# Autodesk Inventor assembly: hologram display version 2 assembly.ipt
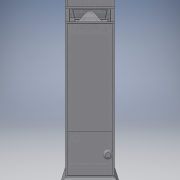
[picture p0: Inventor's stored thumbnail of the model, 180x180]
Saved by Autodesk Inventor 2016 (Build 200138000, 138)
## iProperties
Created: 2017-10-23
Part Number: hologram display version 2 assembly.ipt
Document SubType Name: Assembly
Designer: student
Author: student
## Documents named in this file (13)
- C:\Users\student\Documents\Aaron's Folder\hologram display version 2 assembly.ipt.iam
- C:\Users\student\Documents\Aaron's Folder\base (for assembly).ipt
- C:\Users\student\Documents\Aaron's Folder\support platforms (for assembly).ipt
- C:\Users\student\Documents\Aaron's Folder\side boards (for assembly).ipt
- C:\Users\student\Documents\Aaron's Folder\back board (for assembly).ipt
- C:\Users\student\Documents\Aaron's Folder\front board (for assembly).ipt
- C:\Users\student\Documents\Aaron's Folder\front door (for assembly).ipt
- C:\Users\student\Documents\Aaron's Folder\monitor supports (for assembly).ipt
- C:\Users\student\Documents\Aaron's Folder\monitor frame part1 (for assembly).ipt
- C:\Users\student\Documents\Aaron's Folder\monitor frame part2 (for assembly).ipt
- C:\Users\student\Documents\Aaron's Folder\hologram pyramid (for assembly).ipt
- C:\Users\student\Documents\Aaron's Folder\monitor (for assembly).ipt
- C:\Users\student\Documents\Aaron's Folder\hollow monitor support (for assembly).ipt
## Components (17 placed, 12 different names)
1. base (for assembly):1 — Rigid:1
2. support platforms (for assembly):1 — Rigid:1, Rigid:19, Rigid:29
3. side boards (for assembly):1 — Rigid:18, Rigid:29, Rigid:30
4. side boards (for assembly):2 — Rigid:18
5. support platforms (for assembly):2 — Rigid:19, Rigid:20, Rigid:21, Rigid:22, Rigid:24, Rigid:31
6. back board (for assembly):1 — Rigid:15, Rigid:16, Rigid:30
7. front board (for assembly):1 — Rigid:16
8. front door (for assembly):1 — Rigid:15
9. monitor supports (for assembly):2 — Rigid:21
10. monitor supports (for assembly):3 — Rigid:20, Rigid:25
11. monitor supports (for assembly):4 — Rigid:22
12. hologram pyramid (for assembly):1 — Rigid:24
13. monitor frame part1 (for assembly):1 — Rigid:25, Rigid:27, Rigid:32
14. monitor frame part2 (for assembly):1 — Rigid:32, Rigid:33
15. monitor (for assembly):1 — Rigid:27
16. support platforms (for assembly):3 — Rigid:33
17. hollow monitor support (for assembly):1 — Rigid:31
## Relationships (16: WeldJoint 16)
- Rigid:1 [WeldJoint]: base (for assembly):1 ↔ support platforms (for assembly):1
- Rigid:15 [WeldJoint] (361.95 mm): back board (for assembly):1 ↔ front door (for assembly):1
- Rigid:16 [WeldJoint] (361.95 mm): back board (for assembly):1 ↔ front board (for assembly):1
- Rigid:18 [WeldJoint] (469.9 mm): side boards (for assembly):1 ↔ side boards (for assembly):2
- Rigid:19 [WeldJoint] (1574.8 mm): support platforms (for assembly):1 ↔ support platforms (for assembly):2
- Rigid:20 [WeldJoint]: support platforms (for assembly):2 ↔ monitor supports (for assembly):3
- Rigid:21 [WeldJoint]: support platforms (for assembly):2 ↔ monitor supports (for assembly):2
- Rigid:22 [WeldJoint]: support platforms (for assembly):2 ↔ monitor supports (for assembly):4
- Rigid:24 [WeldJoint] (162.56 mm): support platforms (for assembly):2 ↔ hologram pyramid (for assembly):1
- Rigid:25 [WeldJoint]: monitor supports (for assembly):3 ↔ monitor frame part1 (for assembly):1
- Rigid:27 [WeldJoint]: monitor frame part1 (for assembly):1 ↔ monitor (for assembly):1
- Rigid:29 [WeldJoint]: support platforms (for assembly):1 ↔ side boards (for assembly):1
- Rigid:30 [WeldJoint] (-19.05 mm): side boards (for assembly):1 ↔ back board (for assembly):1
- Rigid:31 [WeldJoint]: support platforms (for assembly):2 ↔ hollow monitor support (for assembly):1
- Rigid:32 [WeldJoint]: monitor frame part1 (for assembly):1 ↔ monitor frame part2 (for assembly):1
- Rigid:33 [WeldJoint]: monitor frame part2 (for assembly):1 ↔ support platforms (for assembly):3
